# Autodesk Inventor assembly: 4xStackBothSides
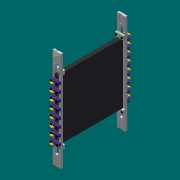
[picture p0: Inventor's stored thumbnail of the model, 180x180]
Saved by Autodesk Inventor 2016 SP1 (Build 200210100, 210)
## iProperties
Created: 2016-02-15
Part Number: 4xStackBothSides
Document SubType Name: Assembly
Designer: sawai
Author: sawai
## Documents named in this file (7)
- C:\Users\sawaiz\OneDrive\projects\scintillatorPanel\4xStackBothSides.iam
- C:\Users\sawaiz\OneDrive\projects\scintillatorPanel\scintillatorPanel.iam
- C:\Users\sawaiz\OneDrive\projects\scintillatorPanel\coluredSpacer.ipt
- C:\Users\sawaiz\OneDrive\projects\scintillatorPanel\mppcMount.ipt
- C:\Users\sawaiz\OneDrive\projects\scintillatorPanel\suppourtBlock.ipt
- C:\Users\sawaiz\OneDrive\projects\scintillatorPanel\4-40x0.5in.ipt
- C:\Users\sawaiz\OneDrive\projects\scintillatorPanel\scintillator.xlsx
## Components (38 placed, 5 different names)
1. mppcMount:1 — Flush:18, Symmetry:7, Mate:3, Mate:4, Mate:5, Mate:7, Flush:21, Symmetry:8, Symmetry:9, Mate:10, Mate:11, Flush:27, Flush:28, Mate:26
2. mppcMount:2 — Flush:18, Symmetry:7, Flush:21, Symmetry:8, Symmetry:9, Mate:8, Flush:23, Mate:12, Mate:13, Flush:26, Flush:29
3. suppourtBlock:1 — Mate:10, Flush:24, Flush:27, Flush:30, Mate:20, Mate:21, Mate:25
4. suppourtBlock:2 — Mate:13, Flush:24, Flush:26, Flush:30, Symmetry:10, Mate:14, Mate:15, Mate:24
5. suppourtBlock:3 — Mate:11, Flush:25, Flush:28, Flush:31, Symmetry:10, Mate:18, Mate:19, Mate:23
6. suppourtBlock:4 — Mate:12, Flush:25, Flush:29, Flush:31, Mate:16, Mate:17, Mate:22, Mate:26
7. 4-40x0.5in:1 — Mate:14, Flush:32
8. 4-40x0.5in:2 — Mate:15, Flush:32, Mate:24
9. 4-40x0.5in:3 — Mate:21, Flush:34
10. 4-40x0.5in:4 — Mate:20, Flush:34, Mate:25
11. 4-40x0.5in:5 — Mate:16, Flush:35
12. 4-40x0.5in:6 — Mate:17, Flush:35, Mate:22
13. 4-40x0.5in:7 — Mate:18, Flush:33, Mate:23
14. 4-40x0.5in:8 — Mate:19, Flush:33
15. scintillatorPanel:1 [sub-assembly] — Mate:3, Mate:4, Mate:5, Mate:6, Flush:20, Mate:9, Flush:22, Flush:23
16. scintillatorPanel:5 [sub-assembly]
17. scintillatorPanel:7 [sub-assembly]
18. scintillatorPanel:8 [sub-assembly]
19. scintillatorPanel:9 [sub-assembly]
20. scintillatorPanel:10 [sub-assembly]
21. scintillatorPanel:11 [sub-assembly]
22. scintillatorPanel:12 [sub-assembly]
23. coluredSpacer:1 — Mate:6, Flush:20, Mate:7
24. coluredSpacer:2
25. coluredSpacer:3
26. coluredSpacer:4
27. coluredSpacer:5
28. coluredSpacer:6
29. coluredSpacer:7
30. coluredSpacer:8
31. scintillatorPanel:4 [sub-assembly] — Mate:8, Mate:9, Flush:22
32. scintillatorPanel:6 [sub-assembly]
33. scintillatorPanel:15 [sub-assembly]
34. scintillatorPanel:16 [sub-assembly]
35. scintillatorPanel:17 [sub-assembly]
36. scintillatorPanel:18 [sub-assembly]
37. scintillatorPanel:19 [sub-assembly]
38. scintillatorPanel:20 [sub-assembly]
## Component patterns: (8 elements, first: scintillatorPanel:1), (8 elements, first: coluredSpacer:1), (8 elements, first: scintillatorPanel:4)
## Relationships (45: Mate 24, Flush 17, Symmetry 4)
- Flush:18: mppcMount:1 ↔ mppcMount:2
- Symmetry:7: mppcMount:1 ↔ mppcMount:2
- Mate:3: mppcMount:1 ↔ scintillatorPanel:1
- Mate:4: mppcMount:1 ↔ scintillatorPanel:1
- Mate:5: mppcMount:1 ↔ scintillatorPanel:1
- Mate:6: scintillatorPanel:1 ↔ coluredSpacer:1
- Flush:20: scintillatorPanel:1 ↔ coluredSpacer:1
- Mate:7: mppcMount:1 ↔ coluredSpacer:1
- Flush:21: mppcMount:1 ↔ mppcMount:2
- Symmetry:8: mppcMount:1 ↔ mppcMount:2
- Symmetry:9: mppcMount:1 ↔ mppcMount:2
- Mate:8: mppcMount:2 ↔ scintillatorPanel:4
- Mate:9: scintillatorPanel:1 ↔ scintillatorPanel:4
- Flush:22: scintillatorPanel:1 ↔ scintillatorPanel:4
- Flush:23: mppcMount:2 ↔ scintillatorPanel:1
- Mate:10: mppcMount:1 ↔ suppourtBlock:1
- Mate:11: mppcMount:1 ↔ suppourtBlock:3
- Mate:12: mppcMount:2 ↔ suppourtBlock:4
- Mate:13: mppcMount:2 ↔ suppourtBlock:2
- Flush:24: suppourtBlock:1 ↔ suppourtBlock:2
- Flush:25: suppourtBlock:3 ↔ suppourtBlock:4
- Flush:26: mppcMount:2 ↔ suppourtBlock:2
- Flush:27: mppcMount:1 ↔ suppourtBlock:1
- Flush:28: mppcMount:1 ↔ suppourtBlock:3
- Flush:29: mppcMount:2 ↔ suppourtBlock:4
- Flush:30: suppourtBlock:1 ↔ suppourtBlock:2
- Flush:31: suppourtBlock:3 ↔ suppourtBlock:4
- Symmetry:10: suppourtBlock:2 ↔ suppourtBlock:3
- Mate:14: suppourtBlock:2 ↔ 4-40x0.5in:1
- Mate:15: suppourtBlock:2 ↔ 4-40x0.5in:2
- Mate:16: suppourtBlock:4 ↔ 4-40x0.5in:5
- Mate:17: suppourtBlock:4 ↔ 4-40x0.5in:6
- Mate:18: suppourtBlock:3 ↔ 4-40x0.5in:7
- Mate:19: suppourtBlock:3 ↔ 4-40x0.5in:8
- Mate:20: suppourtBlock:1 ↔ 4-40x0.5in:4
- Mate:21: suppourtBlock:1 ↔ 4-40x0.5in:3
- Flush:32: 4-40x0.5in:1 ↔ 4-40x0.5in:2
- Flush:33: 4-40x0.5in:7 ↔ 4-40x0.5in:8
- Flush:34: 4-40x0.5in:3 ↔ 4-40x0.5in:4
- Flush:35: 4-40x0.5in:5 ↔ 4-40x0.5in:6
- Mate:22: suppourtBlock:4 ↔ 4-40x0.5in:6
- Mate:23: suppourtBlock:3 ↔ 4-40x0.5in:7
- Mate:24: suppourtBlock:2 ↔ 4-40x0.5in:2
- Mate:25: suppourtBlock:1 ↔ 4-40x0.5in:4
- Mate:26 (-58.672 mm): mppcMount:1 ↔ suppourtBlock:4
## Named parameters: ScintillatorThickness = 10 mm, OpticalFiberClearence = 0.071 mm, ScintillatorEdgeClearence = 3 mm, ScintillatorWidth = 10 mm, ScintillatorHeight = 200 mm, ShallowTrackDepth = 1.142 mm, DeepTrackDepth = 5.571 mm, FiberEdgeOffsett = 5 mm, LoopLargeTrackRatio = 1.1, LoopSmallTrackDiameter = 90 mm, FiberSensorClerence = 0.5 mm, MountingScrewOffsett = 9 mm, LoopLength = 140 mm, silveringThickness = 0.2 mm, rubberizedCoating = 0.0508, mppcMountDepth = 6.35 mm, fingerCount = 16
note: some values were not read from the file. Shown as the stored number, unit unknown: "rubberizedCoating".
